# Autodesk Inventor assembly: Сборка_подлокотник
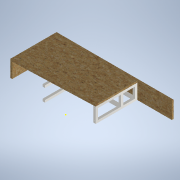
[picture p0: Inventor's stored thumbnail of the model, 180x180]
Saved by Autodesk Inventor 2022 (Build 260153000, 153)
## iProperties
Created: 2021-10-11
Part Number: Сборка_подлокотник
Document SubType Name: Assembly
Designer: Admin
Mass: 8336.05 g
Surface Area: 12825.4 cm^2
Volume: 8336.05 cm^3
Density: 1 g/cm^3
Author: Admin
## Documents named in this file (5)
- C:\Users\Admin\Documents\Сборка_подлокотник.iam
- C:\Users\Admin\Documents\зад.ipt
- C:\Users\Admin\Documents\боковина.ipt
- C:\Users\Admin\Documents\верхушка.ipt
- C:\Users\Admin\Documents\Подлокотник.ipt
## Components (4 placed, 4 different names)
1. зад:1 — Заподлицо:3, Совмещение:3, Заподлицо:4
2. боковина:1 — Совмещение:3, Совмещение:4, Заподлицо:4
3. верхушка:1 — Совмещение:1, Совмещение:2, Заподлицо:3, Совмещение:4
4. Подлокотник:1 — Совмещение:1, Совмещение:2
## Relationships (6: Mate 4, Flush 2)
- Совмещение:1 [Mate]: верхушка:1 ↔ Подлокотник:1
- Совмещение:2 [Mate]: верхушка:1 ↔ Подлокотник:1
- Заподлицо:3 [Flush]: зад:1 ↔ верхушка:1
- Совмещение:3 [Mate]: зад:1 ↔ боковина:1
- Совмещение:4 [Mate]: боковина:1 ↔ верхушка:1
- Заподлицо:4 [Flush]: зад:1 ↔ боковина:1
